# Autodesk Inventor assembly: Burning Table Assembly
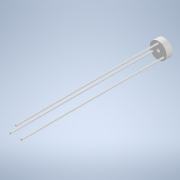
[picture p0: Inventor's stored thumbnail of the model, 180x180]
Saved by Autodesk Inventor 2020 (Build 240168000, 168)
## iProperties
Created: 2019-06-07
Part Number: Burning Table Assembly
Document SubType Name: Assembly
Designer: isadmin
Author: isadmin
## Documents named in this file (3)
- C:\Users\isadmin\Documents\Inventor\IS_2019June01\Burning Table Assembly.iam
- C:\Users\isadmin\Documents\Inventor\IS_2019June01\Burner Table IS v01.ipt
- C:\Users\isadmin\Documents\Inventor\IS_2019June01\Burner Rodx3.ipt
## Components (4 placed, 2 different names)
1. Burner Table IS v01:1 — Insert:1, Insert:2, Insert:3
2. Burner Rodx3:1 — Insert:1
3. Burner Rodx3:2 — Insert:2
4. Burner Rodx3:3 — Insert:3
## Relationships (3: Insert 3)
- Insert:1 (12.7 mm): Burner Table IS v01:1 ↔ Burner Rodx3:1
- Insert:2 (12.7 mm): Burner Table IS v01:1 ↔ Burner Rodx3:2
- Insert:3 (12.7 mm): Burner Table IS v01:1 ↔ Burner Rodx3:3
